# Autodesk Inventor assembly: 000.600 - Третье звездо
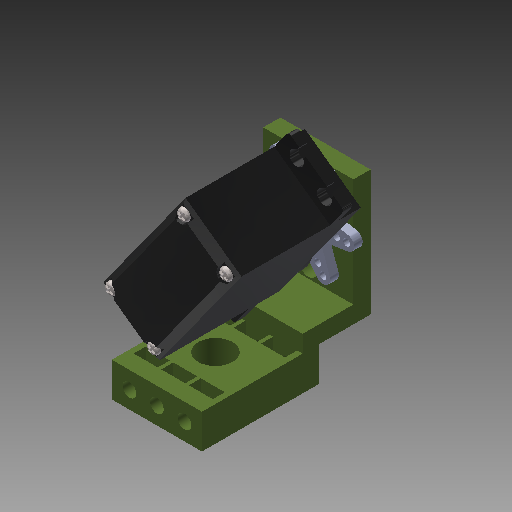
[picture p0: Inventor's stored thumbnail of the model, 512x512]
Saved by Autodesk Inventor 2019 (Build 230136000, 136)
## iProperties
Created: 2020-02-29
Part Number: 000.600 - Третье звездо
Material: Типовые
Document SubType Name: Assembly
Designer: Петров Иван
Author: Петров Иван
## Documents named in this file (4)
- E:\IVAN\Ivan_desktop\GitHub\Manipulation_IRS\hardware\5-DOF\000.600 - Третье звездо.iam
- E:\IVAN\Ivan_desktop\GitHub\Manipulation_IRS\hardware\5-DOF\000.601 - Проставка.ipt
- E:\IVAN\Ivan_desktop\GitHub\Manipulation_IRS\hardware\5-DOF\components\Star Horn MG995.ipt
- E:\IVAN\Ivan_desktop\GitHub\Manipulation_IRS\hardware\5-DOF\components\tower prone.ipt
## Components (3 placed, 3 different names)
1. 000.601 - Проставка:1 — Совмещение:6, Совмещение:7, Совмещение:8
2. Star Horn MG995:1 — Совмещение:4, Совмещение:5, Совмещение:6, Совмещение:7, Совмещение:8
3. tower prone:1 — Совмещение:4, Совмещение:5
## Relationships (5: Mate 5)
- Совмещение:4 [Mate]: Star Horn MG995:1 ↔ tower prone:1
- Совмещение:5 [Mate]: Star Horn MG995:1 ↔ tower prone:1
- Совмещение:6 [Mate]: 000.601 - Проставка:1 ↔ Star Horn MG995:1
- Совмещение:7 [Mate]: 000.601 - Проставка:1 ↔ Star Horn MG995:1
- Совмещение:8 [Mate]: 000.601 - Проставка:1 ↔ Star Horn MG995:1
